# Autodesk Inventor assembly: De truc Z
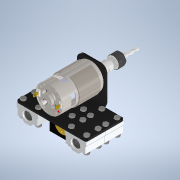
[picture p0: Inventor's stored thumbnail of the model, 180x180]
Saved by Autodesk Inventor 2021 (Build 250183000, 183)
## iProperties
Created: 2021-05-25
Part Number: De truc Z
Document SubType Name: Assembly
Designer: admin
Author: admin
## Documents named in this file (10)
- C:\Users\79449\Documents\CNC_DISENO_DE MAQUINAS\Piezas-Ensambles_Inventor\Segunda_presentación\De truc Z.iam
- C:\Users\79449\Documents\CNC_DISENO_DE MAQUINAS\Piezas-Ensambles_Inventor\Segunda_presentación\SC8uu.ipt
- C:\Users\79449\Documents\CNC_DISENO_DE MAQUINAS\Piezas-Ensambles_Inventor\Segunda_presentación\AoVitmeT8.ipt
- C:\Users\79449\Documents\CNC_DISENO_DE MAQUINAS\Piezas-Ensambles_Inventor\Segunda_presentación\De truc Z chan sat.ipt
- C:\Users\79449\Documents\CNC_DISENO_DE MAQUINAS\Piezas-Ensambles_Inventor\Segunda_presentación\T8 Nut.ipt
- C:\Users\79449\Documents\CNC_DISENO_DE MAQUINAS\Piezas-Ensambles_Inventor\Segunda_presentación\Dong co 775.ipt
- C:\Users\79449\Documents\CNC_DISENO_DE MAQUINAS\Piezas-Ensambles_Inventor\Segunda_presentación\Bo collect ER11\C16-ER11-35L 5mm Shank Chuck Collet.iam
- C:\Users\79449\Documents\Inventor\Content Center Files\R2021\es-ES\AS 1110\AS 1110 - M4 x 12.ipt
- C:\Users\79449\Documents\Inventor\Content Center Files\R2021\es-ES\AS 1110\AS 1110 - M4 x 25.ipt
- C:\Users\79449\Documents\Inventor\Content Center Files\R2021\es-ES\AS 1112 (2)\AS 1112 - M4  Tipo 5.ipt
## Components (47 placed, 9 different names)
1. SC8uu:1 — Mate:11, Mate:12, Mate:13, Coincidencia:129, Coincidencia:131, Coincidencia:133, Coincidencia:135
2. AoVitmeT8:1 — Mate:23, Mate:24, Mate:25, Mate:32, Mate:33
3. SC8uu:2 — Mate:14, Mate:15, Mate:16, Coincidencia:121, Coincidencia:123, Coincidencia:125, Coincidencia:127
4. SC8uu:3 — Mate:17, Mate:18, Mate:19, Coincidencia:137, Coincidencia:139, Coincidencia:149, Coincidencia:151
5. SC8uu:4 — Mate:20, Mate:21, Mate:22, Coincidencia:141, Coincidencia:143, Coincidencia:145, Coincidencia:147
6. De truc Z chan sat:1 — Mate:11, Mate:12, Mate:13, Mate:14, Mate:15, Mate:16, Mate:17, Mate:18, Mate:19, Mate:20, Mate:21, Mate:22, Mate:23, Mate:24, Mate:25, Mate:34, Coincidencia:76, Coincidencia:77, Coincidencia:78, Coincidencia:79, Coincidencia:80, Coincidencia:81, Coincidencia:82, Coincidencia:83, Coincidencia:84, Coincidencia:85, Coincidencia:86, Coincidencia:87, Coincidencia:88, Coincidencia:89, Coincidencia:90, Coincidencia:91, Coincidencia:92, Coincidencia:93, Coincidencia:94, Coincidencia:95, Coincidencia:96, Coincidencia:97, Coincidencia:98, Coincidencia:99, Coincidencia:100, Coincidencia:101, Coincidencia:102, Coincidencia:103, Coincidencia:104, Coincidencia:105, Coincidencia:106, Coincidencia:107, Coincidencia:108, Coincidencia:109, Coincidencia:110, Coincidencia:111, Coincidencia:112, Coincidencia:113, Coincidencia:114, Coincidencia:115, Coincidencia:116, Coincidencia:117, Coincidencia:118, Coincidencia:119
7. Dong co 775:1 — Mate:35
8. T8 Nut:1 — Mate:32, Mate:33
9. C16-ER11-35L 5mm Shank Chuck Collet:1 [sub-assembly] — Mate:34, Mate:35
10. AS 1110 - Métrico M4 x 12:1 — Coincidencia:76, Coincidencia:77
11. AS 1110 - Métrico M4 x 12:2 — Coincidencia:78, Coincidencia:79
12. AS 1110 - Métrico M4 x 25:1 — Coincidencia:80, Coincidencia:81, Coincidencia:122
13. AS 1110 - Métrico M4 x 25:2 — Coincidencia:82, Coincidencia:83
14. AS 1110 - Métrico M4 x 25:3 — Coincidencia:84, Coincidencia:85
15. AS 1110 - Métrico M4 x 25:4 — Coincidencia:86, Coincidencia:87
16. AS 1110 - Métrico M4 x 25:5 — Coincidencia:88, Coincidencia:89
17. AS 1110 - Métrico M4 x 25:6 — Coincidencia:90, Coincidencia:91, Coincidencia:134
18. AS 1110 - Métrico M4 x 25:7 — Coincidencia:92, Coincidencia:93, Coincidencia:132
19. AS 1110 - Métrico M4 x 25:8 — Coincidencia:94, Coincidencia:95, Coincidencia:130
20. AS 1110 - Métrico M4 x 25:9 — Coincidencia:96, Coincidencia:97, Coincidencia:128
21. AS 1110 - Métrico M4 x 25:10 — Coincidencia:98, Coincidencia:99, Coincidencia:126
22. AS 1110 - Métrico M4 x 25:11 — Coincidencia:100, Coincidencia:101, Coincidencia:124
23. AS 1110 - Métrico M4 x 25:12 — Coincidencia:102, Coincidencia:103, Coincidencia:120
24. AS 1110 - Métrico M4 x 25:13 — Coincidencia:104, Coincidencia:105, Coincidencia:136
25. AS 1110 - Métrico M4 x 25:14 — Coincidencia:106, Coincidencia:107, Coincidencia:150
26. AS 1110 - Métrico M4 x 25:15 — Coincidencia:108, Coincidencia:109, Coincidencia:148
27. AS 1110 - Métrico M4 x 25:16 — Coincidencia:110, Coincidencia:111, Coincidencia:138
28. AS 1110 - Métrico M4 x 25:17 — Coincidencia:112, Coincidencia:113, Coincidencia:140
29. AS 1110 - Métrico M4 x 25:18 — Coincidencia:114, Coincidencia:115, Coincidencia:144
30. AS 1110 - Métrico M4 x 25:19 — Coincidencia:116, Coincidencia:117, Coincidencia:146
31. AS 1110 - Métrico M4 x 25:20 — Coincidencia:118, Coincidencia:119, Coincidencia:142
32. AS 1112 (2) - Métrico M4  Tipo 5:1 — Coincidencia:120, Coincidencia:121
33. AS 1112 (2) - Métrico M4  Tipo 5:2 — Coincidencia:122, Coincidencia:123
34. AS 1112 (2) - Métrico M4  Tipo 5:3 — Coincidencia:124, Coincidencia:125
35. AS 1112 (2) - Métrico M4  Tipo 5:4 — Coincidencia:126, Coincidencia:127
36. AS 1112 (2) - Métrico M4  Tipo 5:5 — Coincidencia:128, Coincidencia:129
37. AS 1112 (2) - Métrico M4  Tipo 5:6 — Coincidencia:130, Coincidencia:131
38. AS 1112 (2) - Métrico M4  Tipo 5:7 — Coincidencia:132, Coincidencia:133
39. AS 1112 (2) - Métrico M4  Tipo 5:8 — Coincidencia:134, Coincidencia:135
40. AS 1112 (2) - Métrico M4  Tipo 5:9 — Coincidencia:136, Coincidencia:137
41. AS 1112 (2) - Métrico M4  Tipo 5:10 — Coincidencia:138, Coincidencia:139
42. AS 1112 (2) - Métrico M4  Tipo 5:11 — Coincidencia:140, Coincidencia:141
43. AS 1112 (2) - Métrico M4  Tipo 5:12 — Coincidencia:142, Coincidencia:143
44. AS 1112 (2) - Métrico M4  Tipo 5:13 — Coincidencia:144, Coincidencia:145
45. AS 1112 (2) - Métrico M4  Tipo 5:14 — Coincidencia:146, Coincidencia:147
46. AS 1112 (2) - Métrico M4  Tipo 5:15 — Coincidencia:148, Coincidencia:149
47. AS 1112 (2) - Métrico M4  Tipo 5:16 — Coincidencia:150, Coincidencia:151
## Relationships (97: Mate 97)
- Mate:11: SC8uu:1 ↔ De truc Z chan sat:1
- Mate:12: SC8uu:1 ↔ De truc Z chan sat:1
- Mate:13: SC8uu:1 ↔ De truc Z chan sat:1
- Mate:14: SC8uu:2 ↔ De truc Z chan sat:1
- Mate:15: SC8uu:2 ↔ De truc Z chan sat:1
- Mate:16: SC8uu:2 ↔ De truc Z chan sat:1
- Mate:17: SC8uu:3 ↔ De truc Z chan sat:1
- Mate:18: SC8uu:3 ↔ De truc Z chan sat:1
- Mate:19: SC8uu:3 ↔ De truc Z chan sat:1
- Mate:20: SC8uu:4 ↔ De truc Z chan sat:1
- Mate:21: SC8uu:4 ↔ De truc Z chan sat:1
- Mate:22: SC8uu:4 ↔ De truc Z chan sat:1
- Mate:23: AoVitmeT8:1 ↔ De truc Z chan sat:1
- Mate:24: AoVitmeT8:1 ↔ De truc Z chan sat:1
- Mate:25: AoVitmeT8:1 ↔ De truc Z chan sat:1
- [Mate]: De truc Z chan sat:1 ↔ Dong co 775:1
- [Mate]: De truc Z chan sat:1 ↔ Dong co 775:1
- Mate:32: AoVitmeT8:1 ↔ T8 Nut:1
- Mate:33: AoVitmeT8:1 ↔ T8 Nut:1
- Mate:34 (2 mm): De truc Z chan sat:1 ↔ C16-ER11-35L 5mm Shank Chuck Collet:1
- Mate:35: Dong co 775:1 ↔ C16-ER11-35L 5mm Shank Chuck Collet:1
- Coincidencia:76 [Mate]: De truc Z chan sat:1 ↔ AS 1110 - Métrico M4 x 12:1
- Coincidencia:77 [Mate]: De truc Z chan sat:1 ↔ AS 1110 - Métrico M4 x 12:1
- Coincidencia:78 [Mate]: De truc Z chan sat:1 ↔ AS 1110 - Métrico M4 x 12:2
- Coincidencia:79 [Mate]: De truc Z chan sat:1 ↔ AS 1110 - Métrico M4 x 12:2
- Coincidencia:80 [Mate]: De truc Z chan sat:1 ↔ AS 1110 - Métrico M4 x 25:1
- Coincidencia:81 [Mate]: De truc Z chan sat:1 ↔ AS 1110 - Métrico M4 x 25:1
- Coincidencia:82 [Mate]: De truc Z chan sat:1 ↔ AS 1110 - Métrico M4 x 25:2
- Coincidencia:83 [Mate]: De truc Z chan sat:1 ↔ AS 1110 - Métrico M4 x 25:2
- Coincidencia:84 [Mate]: De truc Z chan sat:1 ↔ AS 1110 - Métrico M4 x 25:3
- Coincidencia:85 [Mate]: De truc Z chan sat:1 ↔ AS 1110 - Métrico M4 x 25:3
- Coincidencia:86 [Mate]: De truc Z chan sat:1 ↔ AS 1110 - Métrico M4 x 25:4
- Coincidencia:87 [Mate]: De truc Z chan sat:1 ↔ AS 1110 - Métrico M4 x 25:4
- Coincidencia:88 [Mate]: De truc Z chan sat:1 ↔ AS 1110 - Métrico M4 x 25:5
- Coincidencia:89 [Mate]: De truc Z chan sat:1 ↔ AS 1110 - Métrico M4 x 25:5
- Coincidencia:90 [Mate]: De truc Z chan sat:1 ↔ AS 1110 - Métrico M4 x 25:6
- Coincidencia:91 [Mate]: De truc Z chan sat:1 ↔ AS 1110 - Métrico M4 x 25:6
- Coincidencia:92 [Mate]: De truc Z chan sat:1 ↔ AS 1110 - Métrico M4 x 25:7
- Coincidencia:93 [Mate]: De truc Z chan sat:1 ↔ AS 1110 - Métrico M4 x 25:7
- Coincidencia:94 [Mate]: De truc Z chan sat:1 ↔ AS 1110 - Métrico M4 x 25:8
- Coincidencia:95 [Mate]: De truc Z chan sat:1 ↔ AS 1110 - Métrico M4 x 25:8
- Coincidencia:96 [Mate]: De truc Z chan sat:1 ↔ AS 1110 - Métrico M4 x 25:9
- Coincidencia:97 [Mate]: De truc Z chan sat:1 ↔ AS 1110 - Métrico M4 x 25:9
- Coincidencia:98 [Mate]: De truc Z chan sat:1 ↔ AS 1110 - Métrico M4 x 25:10
- Coincidencia:99 [Mate]: De truc Z chan sat:1 ↔ AS 1110 - Métrico M4 x 25:10
- Coincidencia:100 [Mate]: De truc Z chan sat:1 ↔ AS 1110 - Métrico M4 x 25:11
- Coincidencia:101 [Mate]: De truc Z chan sat:1 ↔ AS 1110 - Métrico M4 x 25:11
- Coincidencia:102 [Mate]: De truc Z chan sat:1 ↔ AS 1110 - Métrico M4 x 25:12
- Coincidencia:103 [Mate]: De truc Z chan sat:1 ↔ AS 1110 - Métrico M4 x 25:12
- Coincidencia:104 [Mate]: De truc Z chan sat:1 ↔ AS 1110 - Métrico M4 x 25:13
- Coincidencia:105 [Mate]: De truc Z chan sat:1 ↔ AS 1110 - Métrico M4 x 25:13
- Coincidencia:106 [Mate]: De truc Z chan sat:1 ↔ AS 1110 - Métrico M4 x 25:14
- Coincidencia:107 [Mate]: De truc Z chan sat:1 ↔ AS 1110 - Métrico M4 x 25:14
- Coincidencia:108 [Mate]: De truc Z chan sat:1 ↔ AS 1110 - Métrico M4 x 25:15
- Coincidencia:109 [Mate]: De truc Z chan sat:1 ↔ AS 1110 - Métrico M4 x 25:15
- Coincidencia:110 [Mate]: De truc Z chan sat:1 ↔ AS 1110 - Métrico M4 x 25:16
- Coincidencia:111 [Mate]: De truc Z chan sat:1 ↔ AS 1110 - Métrico M4 x 25:16
- Coincidencia:112 [Mate]: De truc Z chan sat:1 ↔ AS 1110 - Métrico M4 x 25:17
- Coincidencia:113 [Mate]: De truc Z chan sat:1 ↔ AS 1110 - Métrico M4 x 25:17
- Coincidencia:114 [Mate]: De truc Z chan sat:1 ↔ AS 1110 - Métrico M4 x 25:18
- Coincidencia:115 [Mate]: De truc Z chan sat:1 ↔ AS 1110 - Métrico M4 x 25:18
- Coincidencia:116 [Mate]: De truc Z chan sat:1 ↔ AS 1110 - Métrico M4 x 25:19
- Coincidencia:117 [Mate]: De truc Z chan sat:1 ↔ AS 1110 - Métrico M4 x 25:19
- Coincidencia:118 [Mate]: De truc Z chan sat:1 ↔ AS 1110 - Métrico M4 x 25:20
- Coincidencia:119 [Mate]: De truc Z chan sat:1 ↔ AS 1110 - Métrico M4 x 25:20
- Coincidencia:120 [Mate]: AS 1110 - Métrico M4 x 25:12 ↔ AS 1112 (2) - Métrico M4  Tipo 5:1
- Coincidencia:121 [Mate]: SC8uu:2 ↔ AS 1112 (2) - Métrico M4  Tipo 5:1
- Coincidencia:122 [Mate]: AS 1110 - Métrico M4 x 25:1 ↔ AS 1112 (2) - Métrico M4  Tipo 5:2
- Coincidencia:123 [Mate]: SC8uu:2 ↔ AS 1112 (2) - Métrico M4  Tipo 5:2
- Coincidencia:124 [Mate]: AS 1110 - Métrico M4 x 25:11 ↔ AS 1112 (2) - Métrico M4  Tipo 5:3
- Coincidencia:125 [Mate]: SC8uu:2 ↔ AS 1112 (2) - Métrico M4  Tipo 5:3
- Coincidencia:126 [Mate]: AS 1110 - Métrico M4 x 25:10 ↔ AS 1112 (2) - Métrico M4  Tipo 5:4
- Coincidencia:127 [Mate]: SC8uu:2 ↔ AS 1112 (2) - Métrico M4  Tipo 5:4
- Coincidencia:128 [Mate]: AS 1110 - Métrico M4 x 25:9 ↔ AS 1112 (2) - Métrico M4  Tipo 5:5
- Coincidencia:129 [Mate]: SC8uu:1 ↔ AS 1112 (2) - Métrico M4  Tipo 5:5
- Coincidencia:130 [Mate]: AS 1110 - Métrico M4 x 25:8 ↔ AS 1112 (2) - Métrico M4  Tipo 5:6
- Coincidencia:131 [Mate]: SC8uu:1 ↔ AS 1112 (2) - Métrico M4  Tipo 5:6
- Coincidencia:132 [Mate]: AS 1110 - Métrico M4 x 25:7 ↔ AS 1112 (2) - Métrico M4  Tipo 5:7
- Coincidencia:133 [Mate]: SC8uu:1 ↔ AS 1112 (2) - Métrico M4  Tipo 5:7
- Coincidencia:134 [Mate]: AS 1110 - Métrico M4 x 25:6 ↔ AS 1112 (2) - Métrico M4  Tipo 5:8
- Coincidencia:135 [Mate]: SC8uu:1 ↔ AS 1112 (2) - Métrico M4  Tipo 5:8
- Coincidencia:136 [Mate]: AS 1110 - Métrico M4 x 25:13 ↔ AS 1112 (2) - Métrico M4  Tipo 5:9
- Coincidencia:137 [Mate]: SC8uu:3 ↔ AS 1112 (2) - Métrico M4  Tipo 5:9
- Coincidencia:138 [Mate]: AS 1110 - Métrico M4 x 25:16 ↔ AS 1112 (2) - Métrico M4  Tipo 5:10
- Coincidencia:139 [Mate]: SC8uu:3 ↔ AS 1112 (2) - Métrico M4  Tipo 5:10
- Coincidencia:140 [Mate]: AS 1110 - Métrico M4 x 25:17 ↔ AS 1112 (2) - Métrico M4  Tipo 5:11
- Coincidencia:141 [Mate]: SC8uu:4 ↔ AS 1112 (2) - Métrico M4  Tipo 5:11
- Coincidencia:142 [Mate]: AS 1110 - Métrico M4 x 25:20 ↔ AS 1112 (2) - Métrico M4  Tipo 5:12
- Coincidencia:143 [Mate]: SC8uu:4 ↔ AS 1112 (2) - Métrico M4  Tipo 5:12
- Coincidencia:144 [Mate]: AS 1110 - Métrico M4 x 25:18 ↔ AS 1112 (2) - Métrico M4  Tipo 5:13
- Coincidencia:145 [Mate]: SC8uu:4 ↔ AS 1112 (2) - Métrico M4  Tipo 5:13
- Coincidencia:146 [Mate]: AS 1110 - Métrico M4 x 25:19 ↔ AS 1112 (2) - Métrico M4  Tipo 5:14
- Coincidencia:147 [Mate]: SC8uu:4 ↔ AS 1112 (2) - Métrico M4  Tipo 5:14
- Coincidencia:148 [Mate]: AS 1110 - Métrico M4 x 25:15 ↔ AS 1112 (2) - Métrico M4  Tipo 5:15
- Coincidencia:149 [Mate]: SC8uu:3 ↔ AS 1112 (2) - Métrico M4  Tipo 5:15
- Coincidencia:150 [Mate]: AS 1110 - Métrico M4 x 25:14 ↔ AS 1112 (2) - Métrico M4  Tipo 5:16
- Coincidencia:151 [Mate]: SC8uu:3 ↔ AS 1112 (2) - Métrico M4  Tipo 5:16
